# Autodesk Inventor assembly: DangoPrinter
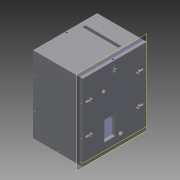
[picture p0: Inventor's stored thumbnail of the model, 180x180]
Saved by Autodesk Inventor 2014 (Build 180170000, 170)
## iProperties
Created: 2014-03-01
Part Number: DangoPrinter
Document SubType Name: Assembly
Designer: Keshuai
Author: Keshuai
## Documents named in this file (10)
- G:\DangoPrinterEnclosure\DangoPrinter.iam
- G:\DangoPrinterEnclosure\print-head-fix.ipt
- G:\DangoPrinterEnclosure\side-right.ipt
- G:\DangoPrinterEnclosure\arduino-fix.ipt
- G:\DangoPrinterEnclosure\drive-fix.ipt
- G:\DangoPrinterEnclosure\face.ipt
- G:\DangoPrinterEnclosure\back.ipt
- G:\DangoPrinterEnclosure\top.ipt
- G:\DangoPrinterEnclosure\left.ipt
- G:\DangoPrinterEnclosure\spacer.ipt
## Components (10 placed, 9 different names)
1. print-head-fix:1 — 表面齐平:1, 表面齐平:11
2. side-right:1 — 表面齐平:1, 表面齐平:2, 配合:1, 表面齐平:3, 表面齐平:4, 表面齐平:5, 表面齐平:6, 表面齐平:7, 表面齐平:8, 表面齐平:10, 配合:6, 表面齐平:12, 表面齐平:13
3. arduino-fix:1 — 表面齐平:2, 配合:1, 表面齐平:3
4. drive-fix:1 — 表面齐平:4
5. face:1 — 表面齐平:5
6. back:1 — 表面齐平:6, 表面齐平:7, 表面齐平:9
7. top:1 — 表面齐平:8
8. top:2 — 表面齐平:9, 表面齐平:10, 配合:6
9. left:1 — 表面齐平:11
10. spacer:1 — 表面齐平:12, 表面齐平:13
## Relationships (15: Flush 13, Mate 2)
- 表面齐平:1 [Flush]: print-head-fix:1 ↔ side-right:1
- 表面齐平:2 [Flush]: side-right:1 ↔ arduino-fix:1
- 配合:1 [Mate]: side-right:1 ↔ arduino-fix:1
- 表面齐平:3 [Flush]: side-right:1 ↔ arduino-fix:1
- 表面齐平:4 [Flush]: side-right:1 ↔ drive-fix:1
- 表面齐平:5 [Flush]: side-right:1 ↔ face:1
- 表面齐平:6 [Flush]: side-right:1 ↔ back:1
- 表面齐平:7 [Flush]: side-right:1 ↔ back:1
- 表面齐平:8 [Flush]: side-right:1 ↔ top:1
- 表面齐平:9 [Flush]: back:1 ↔ top:2
- 表面齐平:10 [Flush]: side-right:1 ↔ top:2
- 配合:6 [Mate]: side-right:1 ↔ top:2
- 表面齐平:11 [Flush]: print-head-fix:1 ↔ left:1
- 表面齐平:12 [Flush]: side-right:1 ↔ spacer:1
- 表面齐平:13 [Flush]: side-right:1 ↔ spacer:1
